# Autodesk Inventor assembly: Assembly1
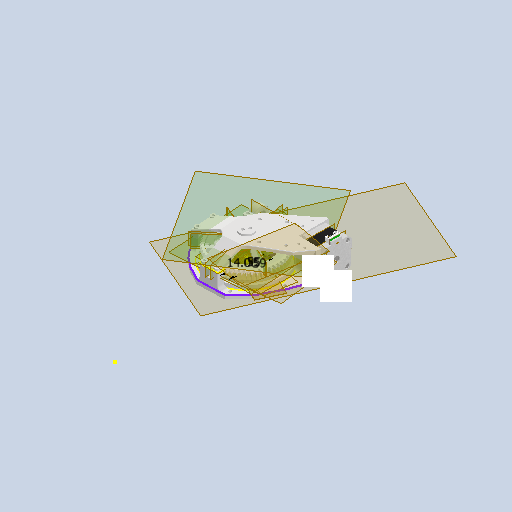
[picture p0: Inventor's stored thumbnail of the model, 512x512]
Saved by Autodesk Inventor 2023.1 (Build 271208000, 208)
## iProperties
Created: 2022-12-24
Part Number: Assembly1
Document SubType Name: Assembly
Designer: USER
Author: USER
## Documents named in this file (7)
- D:\Assembly1.iam
- D:\Assembly1\Design Accelerator\Worm Gears2.iam
- D:\Part48.ipt
- D:\Frame.ipt
- C:\Users\Robot\Downloads\Slideshow\nema-17-stepper-motor-22.snapshot.3\Nema 17 - Busheng 17HD34008-22B\Nema 17 Stepper Motor.iam
- D:\Part3.ipt
- D:\Part5.ipt
## Components (6 placed, 6 different names)
1. Part48:1 — Mate:10, Rotation:2, Flush:16, Flush:17, Flush:18
2. Worm Gears:1 [sub-assembly] — Mate:10, Mate:13, Mate:14, Rotation:2
3. Frame:1 — Flush:14, Mate:11, Mate:12, Mate:14, Flush:15
4. Nema 17 Stepper Motor:1 [sub-assembly] — Mate:11, Mate:12, Mate:13
5. Part3:1 — Flush:13, Flush:15
6. Part5:1 — Flush:16, Flush:17, Flush:18
## Relationships (12: Flush 6, Mate 5, RelateRotation 1)
- Flush:13: Part3:1
- Flush:14 (0.1 mm): Frame:1
- Mate:10: Part48:1 ↔ Worm Gears:1
- Mate:11: Frame:1 ↔ Nema 17 Stepper Motor:1
- Mate:12: Frame:1 ↔ Nema 17 Stepper Motor:1
- Mate:13: Worm Gears:1 ↔ Nema 17 Stepper Motor:1
- Mate:14: Worm Gears:1 ↔ Frame:1
- Rotation:2 [RelateRotation] (1 ul): Part48:1 ↔ Worm Gears:1
- Flush:15 (0.1 mm): Frame:1 ↔ Part3:1
- Flush:16: Part48:1 ↔ Part5:1
- Flush:17 (0.254 mm): Part48:1 ↔ Part5:1
- Flush:18: Part48:1 ↔ Part5:1
